# Autodesk Inventor assembly: Mech Chassis Half v7
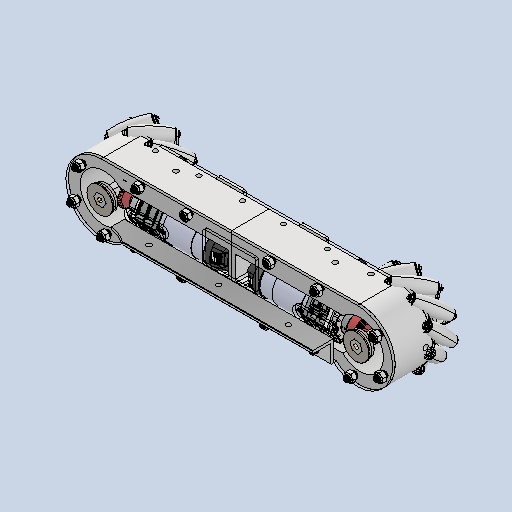
[picture p0: Inventor's stored thumbnail of the model, 512x512]
Saved by Autodesk Inventor 2023 (Build 270158000, 158)
## iProperties
Created: 2021-10-05
Part Number: Mech Chassis Half v7
Document SubType Name: Assembly
Designer: TakeHomePC
Author: TakeHomePC
## Documents named in this file (17)
- C:\Users\matt\Documents\Inventor\FTC\2022-23 FTC\Mech Chassis\Mech Chassis Half v7.iam
- C:\Users\matt\Documents\Inventor\FTC\2022-23 FTC\Mech Chassis\Mech Panel v7 infill_01.ipt
- C:\Users\matt\Documents\Inventor\FTC\2022-23 FTC\Mech Chassis\Mech Motor_Wheel_BevelGears.iam
- C:\Users\matt\Documents\Inventor\FTC\2022-23 FTC\Mech Chassis\Mech Panel v7 infill_01_MIR.ipt
- C:\Users\matt\Documents\Inventor\FTC\2022-23 FTC\Fasteners\M6 x 60.ipt
- C:\Users\matt\Documents\Inventor\FTC\2022-23 FTC\Fasteners\M5 Flanged Nut.ipt
- C:\Users\matt\Documents\Inventor\FTC\2022-23 FTC\Mech Chassis\Mech Panel v7 skin exterior.ipt
- C:\Users\matt\Documents\Inventor\FTC\2022-23 FTC\Mech Chassis\Mech Panel v7 skin interior.ipt
- C:\Users\matt\Documents\Inventor\FTC\2022-23 FTC\Mech Chassis\am-2986 FR8ZZ Hex Bearing (1).ipt
- C:\Users\matt\Documents\Inventor\FTC\2022-23 FTC\Fasteners\M6 x 10.ipt
- C:\Users\matt\Documents\Inventor\FTC\2022-23 FTC\Mech Chassis\Mech Wheel and Bearings.iam
- C:\Users\matt\Documents\Inventor\FTC\2022-23 FTC\Mech Chassis\Mech Motor_Wheel.iam
- C:\Users\matt\Documents\Inventor\FTC\2022-23 FTC\Mech Chassis\am-3772 1.25, 20T, 500 Hex Bore.ipt
- C:\Users\matt\Documents\Inventor\FTC\2022-23 FTC\Mech Chassis\Motor Cleat.ipt
- C:\Users\matt\Documents\Inventor\FTC\2022-23 FTC\Fasteners\M6 Nut.ipt
- C:\Users\matt\Documents\Inventor\FTC\2022-23 FTC\Mech Chassis\1in Angle x 250.ipt
- C:\Users\matt\Documents\Inventor\FTC\2022-23 FTC\Fasteners\M6 x 65.ipt
## Components (51 placed, 16 different names)
1. Mech Motor_Wheel_BevelGears:1 [sub-assembly] — Mate:1, Mate:88, Mate:89, Mate:90, Angle:2
2. Mech Motor_Wheel_BevelGears:2 [sub-assembly] — Mate:1, Mate:103, Mate:105, Mate:106, Mate:120
3. Mech Panel v7 infill_01:1 — Flush:9, Flush:10, Mate:52, Mate:56, Mate:57, Mate:58, Flush:18, Mate:174, Mate:183
4. Mech Panel v7 infill_01_MIR:1 — Flush:9, Flush:10, Mate:52, Flush:17, Mate:165, Angle:2, Mate:226, Mate:251
5. M5 Flanged Nut:1
6. Mech Panel v7 skin exterior:2 — Mate:56, Mate:57, Mate:81, Mate:82, Mate:100, Mate:101, Mate:241, Mate:242, Mate:243, Mate:244, Mate:245, Mate:246, Mate:247, Mate:248, Mate:249, Mate:250, Mate:257
7. Mech Panel v7 skin interior:1 — Mate:58, Mate:69, Mate:70, Mate:78, Mate:79, Mate:118, Mate:119, Mate:184, Mate:194, Mate:195, Mate:196, Mate:197, Mate:198, Mate:199, Mate:200, Mate:201, Mate:202, Mate:203, Mate:204, Mate:205, Mate:206, Mate:207, Mate:208, Mate:252
8. am-2986 FR8ZZ Hex Bearing (1):1 — Mate:69, Mate:70, Mate:85, Mate:87, Mate:173, Mate:226
9. am-2986 FR8ZZ Hex Bearing (1):2 — Mate:78, Mate:79, Mate:102, Mate:104, Mate:180
10. M6 x 10:2 — Mate:176
11. Mech Wheel and Bearings:1 [sub-assembly]
12. Mech Motor_Wheel:1 [sub-assembly] — Mate:173, Flush:26, Mate:260
13. am-2986 FR8ZZ Hex Bearing (1):3 — Mate:81, Mate:82, Mate:165, Mate:169, Flush:26
14. am-3772 1.25, 20T, 500 Hex Bore:1 — Mate:85, Mate:88, Mate:260
15. am-3772 1.25, 20T, 500 Hex Bore:2 — Mate:87, Mate:89, Mate:90
16. Mech Motor_Wheel:2 [sub-assembly] — Mate:174, Flush:27, Mate:175, Mate:176, Mate:181, Mate:182
17. am-2986 FR8ZZ Hex Bearing (1):5 — Mate:100, Mate:101, Flush:27, Mate:175
18. am-3772 1.25, 20T, 500 Hex Bore:3 — Mate:102, Mate:103, Mate:180, Mate:181
19. am-3772 1.25, 20T, 500 Hex Bore:4 — Mate:104, Mate:105, Mate:106, Mate:182
20. Motor Cleat:1 — Mate:118, Mate:120, Flush:18, Mate:189, Mate:190, Mate:264
21. Motor Cleat:2 — Mate:119, Flush:17, Mate:191, Mate:192, Mate:261, Mate:262
22. M6 x 10:3 — Mate:169
23. M6 x 60:1 — Mate:183, Mate:184, Mate:228, Mate:259
24. M6 x 60:2 — Mate:199, Mate:200, Mate:236
25. M6 x 60:3 — Mate:197, Mate:198, Mate:238
26. M6 x 60:4 — Mate:189, Mate:190, Mate:233
27. M6 x 60:5 — Mate:201, Mate:202, Mate:232
28. M6 Nut:2 — Mate:232, Mate:244
29. M6 x 60:6 — Mate:203, Mate:204, Mate:231
30. M6 x 60:7 — Mate:205, Mate:206, Mate:229
31. M6 x 60:8 — Mate:207, Mate:208, Mate:230
32. M6 x 60:9 — Mate:194, Mate:235
33. M6 x 60:10 — Mate:195, Mate:196, Mate:237
34. M6 x 60:11 — Mate:191, Mate:192, Mate:234
35. M6 Nut:3 — Mate:233, Mate:245
36. M6 Nut:4 — Mate:231, Mate:243
37. M6 Nut:6 — Mate:234, Mate:246
38. M6 Nut:7 — Mate:235, Mate:247
39. M6 Nut:8 — Mate:236, Mate:248
40. M6 Nut:9 — Mate:238, Mate:250
41. M6 Nut:10 — Mate:237, Mate:249
42. M6 Nut:12 — Mate:229, Mate:242
43. M6 Nut:13 — Mate:230, Mate:241
44. M6 Nut:14 — Mate:228
45. 1in Angle x 250:1 — Mate:257, Mate:258, Mate:259, Mate:263, Mate:267, Mate:268, Mate:269
46. M6 x 60:14 — Mate:251, Mate:252, Mate:253
47. M6 Nut:15 — Mate:253, Mate:258
48. M6 x 65:1 — Mate:261, Mate:262, Mate:266, Mate:267
49. M6 x 65:2 — Mate:263, Mate:264, Mate:265
50. M6 Nut:16 — Mate:266, Mate:268
51. M6 Nut:17 — Mate:265, Mate:269
## Relationships (101: Mate 94, Flush 6, Angle 1)
- Mate:1: Mech Motor_Wheel_BevelGears:1 ↔ Mech Motor_Wheel_BevelGears:2
- Flush:9: Mech Panel v7 infill_01:1 ↔ Mech Panel v7 infill_01_MIR:1
- Flush:10: Mech Panel v7 infill_01:1 ↔ Mech Panel v7 infill_01_MIR:1
- Mate:52: Mech Panel v7 infill_01:1 ↔ Mech Panel v7 infill_01_MIR:1
- Mate:56: Mech Panel v7 infill_01:1 ↔ Mech Panel v7 skin exterior:2
- Mate:57: Mech Panel v7 infill_01:1 ↔ Mech Panel v7 skin exterior:2
- Mate:58: Mech Panel v7 infill_01:1 ↔ Mech Panel v7 skin interior:1
- Mate:69: Mech Panel v7 skin interior:1 ↔ am-2986 FR8ZZ Hex Bearing (1):1
- Mate:70: Mech Panel v7 skin interior:1 ↔ am-2986 FR8ZZ Hex Bearing (1):1
- Mate:78: Mech Panel v7 skin interior:1 ↔ am-2986 FR8ZZ Hex Bearing (1):2
- Mate:79: Mech Panel v7 skin interior:1 ↔ am-2986 FR8ZZ Hex Bearing (1):2
- Mate:81: Mech Panel v7 skin exterior:2 ↔ am-2986 FR8ZZ Hex Bearing (1):3
- Mate:82: Mech Panel v7 skin exterior:2 ↔ am-2986 FR8ZZ Hex Bearing (1):3
- Mate:85: am-2986 FR8ZZ Hex Bearing (1):1 ↔ am-3772 1.25, 20T, 500 Hex Bore:1
- Mate:87 (23.114 mm): am-2986 FR8ZZ Hex Bearing (1):1 ↔ am-3772 1.25, 20T, 500 Hex Bore:2
- Mate:88 (23.114 mm): Mech Motor_Wheel_BevelGears:1 ↔ am-3772 1.25, 20T, 500 Hex Bore:1
- Mate:89: Mech Motor_Wheel_BevelGears:1 ↔ am-3772 1.25, 20T, 500 Hex Bore:2
- Mate:90: Mech Motor_Wheel_BevelGears:1 ↔ am-3772 1.25, 20T, 500 Hex Bore:2
- Mate:100: Mech Panel v7 skin exterior:2 ↔ am-2986 FR8ZZ Hex Bearing (1):5
- Mate:101: Mech Panel v7 skin exterior:2 ↔ am-2986 FR8ZZ Hex Bearing (1):5
- Mate:102: am-2986 FR8ZZ Hex Bearing (1):2 ↔ am-3772 1.25, 20T, 500 Hex Bore:3
- Mate:103 (23.114 mm): Mech Motor_Wheel_BevelGears:2 ↔ am-3772 1.25, 20T, 500 Hex Bore:3
- Mate:104 (23.114 mm): am-2986 FR8ZZ Hex Bearing (1):2 ↔ am-3772 1.25, 20T, 500 Hex Bore:4
- Mate:105: Mech Motor_Wheel_BevelGears:2 ↔ am-3772 1.25, 20T, 500 Hex Bore:4
- Mate:106: Mech Motor_Wheel_BevelGears:2 ↔ am-3772 1.25, 20T, 500 Hex Bore:4
- Mate:118: Mech Panel v7 skin interior:1 ↔ Motor Cleat:1
- Mate:119: Mech Panel v7 skin interior:1 ↔ Motor Cleat:2
- Flush:17: Mech Panel v7 infill_01_MIR:1 ↔ Motor Cleat:2
- Mate:120: Mech Motor_Wheel_BevelGears:2 ↔ Motor Cleat:1
- Flush:18: Mech Panel v7 infill_01:1 ↔ Motor Cleat:1
- Mate:165: Mech Panel v7 infill_01_MIR:1 ↔ am-2986 FR8ZZ Hex Bearing (1):3
- Angle:2 (0 deg): Mech Motor_Wheel_BevelGears:1 ↔ Mech Panel v7 infill_01_MIR:1
- Mate:169: am-2986 FR8ZZ Hex Bearing (1):3 ↔ M6 x 10:3
- Mate:173: am-2986 FR8ZZ Hex Bearing (1):1 ↔ Mech Motor_Wheel:1
- Flush:26: Mech Motor_Wheel:1 ↔ am-2986 FR8ZZ Hex Bearing (1):3
- Mate:174: Mech Panel v7 infill_01:1 ↔ Mech Motor_Wheel:2
- Flush:27: Mech Motor_Wheel:2 ↔ am-2986 FR8ZZ Hex Bearing (1):5
- Mate:175: Mech Motor_Wheel:2 ↔ am-2986 FR8ZZ Hex Bearing (1):5
- Mate:176: M6 x 10:2 ↔ Mech Motor_Wheel:2
- Mate:180: am-2986 FR8ZZ Hex Bearing (1):2 ↔ am-3772 1.25, 20T, 500 Hex Bore:3
- Mate:181: Mech Motor_Wheel:2 ↔ am-3772 1.25, 20T, 500 Hex Bore:3
- Mate:182: Mech Motor_Wheel:2 ↔ am-3772 1.25, 20T, 500 Hex Bore:4
- Mate:183: Mech Panel v7 infill_01:1 ↔ M6 x 60:1
- Mate:184: Mech Panel v7 skin interior:1 ↔ M6 x 60:1
- Mate:189: Motor Cleat:1 ↔ M6 x 60:4
- Mate:190: Motor Cleat:1 ↔ M6 x 60:4
- Mate:191: Motor Cleat:2 ↔ M6 x 60:11
- Mate:192: Motor Cleat:2 ↔ M6 x 60:11
- Mate:194: Mech Panel v7 skin interior:1 ↔ M6 x 60:9
- Mate:195: Mech Panel v7 skin interior:1 ↔ M6 x 60:10
- Mate:196: Mech Panel v7 skin interior:1 ↔ M6 x 60:10
- Mate:197: Mech Panel v7 skin interior:1 ↔ M6 x 60:3
- Mate:198: Mech Panel v7 skin interior:1 ↔ M6 x 60:3
- Mate:199: Mech Panel v7 skin interior:1 ↔ M6 x 60:2
- Mate:200: Mech Panel v7 skin interior:1 ↔ M6 x 60:2
- Mate:201: Mech Panel v7 skin interior:1 ↔ M6 x 60:5
- Mate:202: Mech Panel v7 skin interior:1 ↔ M6 x 60:5
- Mate:203: Mech Panel v7 skin interior:1 ↔ M6 x 60:6
- Mate:204: Mech Panel v7 skin interior:1 ↔ M6 x 60:6
- Mate:205: Mech Panel v7 skin interior:1 ↔ M6 x 60:7
- Mate:206: Mech Panel v7 skin interior:1 ↔ M6 x 60:7
- Mate:207: Mech Panel v7 skin interior:1 ↔ M6 x 60:8
- Mate:208: Mech Panel v7 skin interior:1 ↔ M6 x 60:8
- Mate:226: Mech Panel v7 infill_01_MIR:1 ↔ am-2986 FR8ZZ Hex Bearing (1):1
- Mate:228: M6 x 60:1 ↔ M6 Nut:14
- Mate:229: M6 x 60:7 ↔ M6 Nut:12
- Mate:230: M6 x 60:8 ↔ M6 Nut:13
- Mate:231: M6 x 60:6 ↔ M6 Nut:4
- Mate:232: M6 x 60:5 ↔ M6 Nut:2
- Mate:233: M6 x 60:4 ↔ M6 Nut:3
- Mate:234: M6 x 60:11 ↔ M6 Nut:6
- Mate:235: M6 x 60:9 ↔ M6 Nut:7
- Mate:236: M6 x 60:2 ↔ M6 Nut:8
- Mate:237: M6 x 60:10 ↔ M6 Nut:10
- Mate:238: M6 x 60:3 ↔ M6 Nut:9
- Mate:241: Mech Panel v7 skin exterior:2 ↔ M6 Nut:13
- Mate:242: Mech Panel v7 skin exterior:2 ↔ M6 Nut:12
- Mate:243: Mech Panel v7 skin exterior:2 ↔ M6 Nut:4
- Mate:244: Mech Panel v7 skin exterior:2 ↔ M6 Nut:2
- Mate:245: Mech Panel v7 skin exterior:2 ↔ M6 Nut:3
- Mate:246: Mech Panel v7 skin exterior:2 ↔ M6 Nut:6
- Mate:247: Mech Panel v7 skin exterior:2 ↔ M6 Nut:7
- Mate:248: Mech Panel v7 skin exterior:2 ↔ M6 Nut:8
- Mate:249: Mech Panel v7 skin exterior:2 ↔ M6 Nut:10
- Mate:250: Mech Panel v7 skin exterior:2 ↔ M6 Nut:9
- Mate:251: Mech Panel v7 infill_01_MIR:1 ↔ M6 x 60:14
- Mate:252: Mech Panel v7 skin interior:1 ↔ M6 x 60:14
- Mate:253: M6 x 60:14 ↔ M6 Nut:15
- Mate:257: Mech Panel v7 skin exterior:2 ↔ 1in Angle x 250:1
- Mate:258: 1in Angle x 250:1 ↔ M6 Nut:15
- Mate:259: M6 x 60:1 ↔ 1in Angle x 250:1
- Mate:260: Mech Motor_Wheel:1 ↔ am-3772 1.25, 20T, 500 Hex Bore:1
- Mate:261: Motor Cleat:2 ↔ M6 x 65:1
- Mate:262: Motor Cleat:2 ↔ M6 x 65:1
- Mate:263: 1in Angle x 250:1 ↔ M6 x 65:2
- Mate:264: Motor Cleat:1 ↔ M6 x 65:2
- Mate:265: M6 x 65:2 ↔ M6 Nut:17
- Mate:266: M6 x 65:1 ↔ M6 Nut:16
- Mate:267: 1in Angle x 250:1 ↔ M6 x 65:1
- Mate:268: 1in Angle x 250:1 ↔ M6 Nut:16
- Mate:269: 1in Angle x 250:1 ↔ M6 Nut:17
